# Autodesk Inventor assembly: Kraken-MarkQ.2
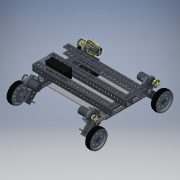
[picture p0: Inventor's stored thumbnail of the model, 180x180]
Saved by Autodesk Inventor 2016 (Build 200138000, 138)
## iProperties
Created: 2015-09-01
Part Number: Kraken-MarkQ.2
Document SubType Name: Assembly
Designer: Tim
Author: Tim
## Documents named in this file (15)
- C:\Users\Tim\Documents\GitHub\phi_robotics\3d-models\FTC_Tetrix_KOP_Block_Party\Tim Bloot Designs\Kraken-MarkQ.2.iam
- C:\Users\Tim\Documents\GitHub\phi_robotics\3d-models\FTC_Tetrix_KOP_Block_Party\Tetrix_Kit_FTC\Autodesk Inventor Files\tetrix_angle-288 MM.ipt
- C:\Users\Tim\Documents\GitHub\phi_robotics\3d-models\FTC_Tetrix_KOP_Block_Party\Tetrix_Kit_FTC\Autodesk Inventor Files\tetrix_flat_bar-288 MM.ipt
- C:\Users\Tim\Documents\GitHub\phi_robotics\3d-models\FTC_Tetrix_KOP_Block_Party\Tetrix_Kit_FTC\Autodesk Inventor Files\tetrix_c_channel-2.ipt
- C:\Users\Tim\Documents\GitHub\phi_robotics\3d-models\FTC_Tetrix_KOP_Block_Party\Tim Bloot Designs\tetrix_739376_2pc_motormnt_2013.iam
- C:\Users\Tim\Documents\GitHub\phi_robotics\3d-models\FTC_Tetrix_KOP_Block_Party\Tetrix_Kit_FTC\Autodesk Inventor Files\tetrix_bushing.ipt
- C:\Users\Tim\Documents\GitHub\phi_robotics\3d-models\FTC_Tetrix_KOP_Block_Party\WheelNChainGear.iam
- C:\Users\Tim\Documents\GitHub\phi_robotics\3d-models\FTC_Tetrix_KOP_Block_Party\Tetrix_Kit_FTC\Autodesk Inventor Files\tetrix_motor.iam
- C:\Users\Tim\Documents\GitHub\phi_robotics\3d-models\FTC_Tetrix_KOP_Block_Party\Tetrix_Kit_FTC\Autodesk Inventor Files\tetrix_c_channel-5.ipt
- C:\Users\Tim\Documents\GitHub\phi_robotics\3d-models\FTC_Tetrix_KOP_Block_Party\Tim Bloot Designs\SmallCGearN'MLock.iam
- C:\Users\Tim\Documents\GitHub\phi_robotics\3d-models\FTC_Tetrix_KOP_Block_Party\Tim Bloot Designs\KrackenPlate1.ipt
- C:\Users\Tim\Documents\GitHub\phi_robotics\3d-models\FTC_Tetrix_KOP_Block_Party\Tetrix_Kit_FTC\Autodesk Inventor Files\tetrix_motor_controller.ipt
- C:\Users\Tim\Documents\GitHub\phi_robotics\3d-models\FTC_Tetrix_KOP_Block_Party\Tetrix_Kit_FTC\Autodesk Inventor Files\tetrix_c_channel-round.ipt
- C:\Users\Tim\Documents\GitHub\phi_robotics\3d-models\FTC_Tetrix_KOP_Block_Party\Tetrix_Kit_FTC\Autodesk Inventor Files\tetrix_batterypack.ipt
- C:\Users\Tim\Documents\GitHub\phi_robotics\3d-models\FTC_Tetrix_KOP_Block_Party\Tetrix_Kit_FTC\Autodesk Inventor Files\tetrix_bat_pack_brkt.ipt
## Components (49 placed, 14 different names)
1. tetrix_angle-288 MM:1 — Rigid:20, Rigid:21, Rigid:34, Rigid:38, Rigid:39
2. tetrix_angle-288 MM:2 — Rigid:23, Rigid:24, Rigid:35, Rigid:41, Rigid:42
3. tetrix_flat_bar-288 MM:1 — Rigid:7, Rigid:8
4. tetrix_flat_bar-288 MM:2 — Rigid:3, Rigid:4
5. tetrix_c_channel-2:1 — Rigid:3, Rigid:11, Rotational:2, Rotational:3, Rigid:21
6. tetrix_c_channel-2:2 — Rigid:7, Rigid:18, Rigid:24, Rotational:13, Rotational:14
7. tetrix_c_channel-2:3 — Rigid:8, Rigid:13, Rigid:23, Rotational:10, Rotational:11
8. tetrix_c_channel-2:4 — Rigid:4, Rotational:5, Rotational:6, Rigid:12, Rigid:20
9. tetrix_739376_2pc_motormnt_2013:1 [sub-assembly] — Rigid:11, Rotational:8
10. tetrix_739376_2pc_motormnt_2013:2 [sub-assembly] — Rigid:12, Rotational:9
11. tetrix_bushing:1 — Rotational:2
12. tetrix_bushing:2 — Rotational:3, Rotational:4
13. WheelNChainGear:1 [sub-assembly] — Rotational:4
14. WheelNChainGear:2 [sub-assembly] — Rotational:7
15. tetrix_bushing:3 — Rotational:6
16. tetrix_bushing:4 — Rotational:5, Rotational:7
17. tetrix_739376_2pc_motormnt_2013:3 [sub-assembly] — Rigid:13, Rotational:16
18. tetrix_739376_2pc_motormnt_2013:4 [sub-assembly] — Rigid:18, Rotational:17
19. tetrix_motor:1 [sub-assembly] — Rotational:8, Rigid:32
20. tetrix_motor:2 [sub-assembly] — Rotational:9, Rigid:33
21. WheelNChainGear:3 [sub-assembly] — Rotational:15
22. WheelNChainGear:4 [sub-assembly] — Rotational:12
23. tetrix_bushing:5 — Rotational:10, Rotational:12
24. tetrix_bushing:6 — Rotational:11
25. tetrix_c_channel-5:1 — Rigid:43, Rigid:44
26. tetrix_bushing:7 — Rotational:14, Rotational:15
27. tetrix_bushing:8 — Rotational:13
28. SmallCGearN'MLock:1 [sub-assembly] — Rigid:32
29. SmallCGearN'MLock:2 [sub-assembly] — Rigid:33
30. KrackenPlate1:1 — Rigid:34, Rigid:35, Mate:1
31. tetrix_motor_controller:1 — Mate:1
32. tetrix_motor:3 [sub-assembly] — Rotational:16, Rigid:36
33. tetrix_motor:4 [sub-assembly] — Rotational:17, Rigid:37
34. SmallCGearN'MLock:3 [sub-assembly] — Rigid:37
35. SmallCGearN'MLock:4 [sub-assembly] — Rigid:36
36. tetrix_c_channel-2:5 — Rigid:42, Rigid:43, Rigid:50, Rigid:57
37. tetrix_c_channel-2:6 — Rigid:41, Rigid:46, Rigid:47
38. tetrix_c_channel-2:7 — Rigid:39, Rigid:44, Rigid:49, Rigid:55
39. tetrix_c_channel-2:8 — Rigid:38, Rigid:45, Rigid:48
40. tetrix_c_channel-5:2 — Rigid:45, Rigid:46
41. tetrix_c_channel-round:1 — Rigid:47
42. tetrix_c_channel-round:2 — Rigid:48
43. tetrix_c_channel-round:3 — Rigid:49
44. tetrix_c_channel-round:4 — Rigid:50
45. tetrix_c_channel-5:3 — Rigid:54, Rigid:56
46. tetrix_c_channel-round:5 — Rigid:54, Rigid:55
47. tetrix_c_channel-round:6 — Rigid:56, Rigid:57
48. tetrix_batterypack:2
49. tetrix_bat_pack_brkt:1
## Relationships (51: WeldJoint 34, RevoluteJoint 16, Mate 1)
- Rigid:3 [WeldJoint]: tetrix_flat_bar-288 MM:2 ↔ tetrix_c_channel-2:1
- Rigid:4 [WeldJoint]: tetrix_flat_bar-288 MM:2 ↔ tetrix_c_channel-2:4
- Rigid:7 [WeldJoint]: tetrix_flat_bar-288 MM:1 ↔ tetrix_c_channel-2:2
- Rigid:8 [WeldJoint]: tetrix_flat_bar-288 MM:1 ↔ tetrix_c_channel-2:3
- Rigid:11 [WeldJoint]: tetrix_c_channel-2:1 ↔ tetrix_739376_2pc_motormnt_2013:1
- Rotational:2 [RevoluteJoint]: tetrix_c_channel-2:1 ↔ tetrix_bushing:1
- Rotational:3 [RevoluteJoint]: tetrix_c_channel-2:1 ↔ tetrix_bushing:2
- Rotational:4 [RevoluteJoint] (-25 mm): tetrix_bushing:2 ↔ WheelNChainGear:1
- Rotational:5 [RevoluteJoint]: tetrix_c_channel-2:4 ↔ tetrix_bushing:4
- Rotational:6 [RevoluteJoint]: tetrix_c_channel-2:4 ↔ tetrix_bushing:3
- Rotational:7 [RevoluteJoint] (-25 mm): WheelNChainGear:2 ↔ tetrix_bushing:4
- Rigid:12 [WeldJoint]: tetrix_c_channel-2:4 ↔ tetrix_739376_2pc_motormnt_2013:2
- Rigid:13 [WeldJoint]: tetrix_c_channel-2:3 ↔ tetrix_739376_2pc_motormnt_2013:3
- Rotational:8 [RevoluteJoint]: tetrix_739376_2pc_motormnt_2013:1 ↔ tetrix_motor:1
- Rotational:9 [RevoluteJoint]: tetrix_739376_2pc_motormnt_2013:2 ↔ tetrix_motor:2
- Rigid:18 [WeldJoint]: tetrix_c_channel-2:2 ↔ tetrix_739376_2pc_motormnt_2013:4
- Rigid:20 [WeldJoint]: tetrix_angle-288 MM:1 ↔ tetrix_c_channel-2:4
- Rigid:21 [WeldJoint]: tetrix_angle-288 MM:1 ↔ tetrix_c_channel-2:1
- Rigid:23 [WeldJoint]: tetrix_angle-288 MM:2 ↔ tetrix_c_channel-2:3
- Rigid:24 [WeldJoint]: tetrix_angle-288 MM:2 ↔ tetrix_c_channel-2:2
- Rotational:10 [RevoluteJoint]: tetrix_c_channel-2:3 ↔ tetrix_bushing:5
- Rotational:11 [RevoluteJoint]: tetrix_c_channel-2:3 ↔ tetrix_bushing:6
- Rotational:12 [RevoluteJoint] (-25 mm): WheelNChainGear:4 ↔ tetrix_bushing:5
- Rotational:13 [RevoluteJoint]: tetrix_c_channel-2:2 ↔ tetrix_bushing:8
- Rotational:14 [RevoluteJoint]: tetrix_c_channel-2:2 ↔ tetrix_bushing:7
- Rotational:15 [RevoluteJoint] (-25 mm): WheelNChainGear:3 ↔ tetrix_bushing:7
- Rigid:32 [WeldJoint] (-11.5 mm): tetrix_motor:1 ↔ SmallCGearN'MLock:1
- Rigid:33 [WeldJoint] (-11.5 mm): tetrix_motor:2 ↔ SmallCGearN'MLock:2
- Rigid:34 [WeldJoint]: tetrix_angle-288 MM:1 ↔ KrackenPlate1:1
- Rigid:35 [WeldJoint]: tetrix_angle-288 MM:2 ↔ KrackenPlate1:1
- Mate:1: KrackenPlate1:1 ↔ tetrix_motor_controller:1
- Rotational:16 [RevoluteJoint]: tetrix_739376_2pc_motormnt_2013:3 ↔ tetrix_motor:3
- Rotational:17 [RevoluteJoint]: tetrix_739376_2pc_motormnt_2013:4 ↔ tetrix_motor:4
- Rigid:36 [WeldJoint] (-11.5 mm): tetrix_motor:3 ↔ SmallCGearN'MLock:4
- Rigid:37 [WeldJoint]: tetrix_motor:4 ↔ SmallCGearN'MLock:3
- Rigid:38 [WeldJoint]: tetrix_angle-288 MM:1 ↔ tetrix_c_channel-2:8
- Rigid:39 [WeldJoint]: tetrix_angle-288 MM:1 ↔ tetrix_c_channel-2:7
- Rigid:41 [WeldJoint]: tetrix_angle-288 MM:2 ↔ tetrix_c_channel-2:6
- Rigid:42 [WeldJoint]: tetrix_angle-288 MM:2 ↔ tetrix_c_channel-2:5
- Rigid:43 [WeldJoint]: tetrix_c_channel-5:1 ↔ tetrix_c_channel-2:5
- Rigid:44 [WeldJoint]: tetrix_c_channel-5:1 ↔ tetrix_c_channel-2:7
- Rigid:45 [WeldJoint]: tetrix_c_channel-2:8 ↔ tetrix_c_channel-5:2
- Rigid:46 [WeldJoint]: tetrix_c_channel-2:6 ↔ tetrix_c_channel-5:2
- Rigid:47 [WeldJoint]: tetrix_c_channel-2:6 ↔ tetrix_c_channel-round:1
- Rigid:48 [WeldJoint]: tetrix_c_channel-2:8 ↔ tetrix_c_channel-round:2
- Rigid:49 [WeldJoint]: tetrix_c_channel-2:7 ↔ tetrix_c_channel-round:3
- Rigid:50 [WeldJoint]: tetrix_c_channel-2:5 ↔ tetrix_c_channel-round:4
- Rigid:54 [WeldJoint]: tetrix_c_channel-5:3 ↔ tetrix_c_channel-round:5
- Rigid:55 [WeldJoint] (-0.25 mm): tetrix_c_channel-2:7 ↔ tetrix_c_channel-round:5
- Rigid:56 [WeldJoint]: tetrix_c_channel-5:3 ↔ tetrix_c_channel-round:6
- Rigid:57 [WeldJoint] (0.25 mm): tetrix_c_channel-2:5 ↔ tetrix_c_channel-round:6
